# Autodesk Inventor assembly: SpacingStrut
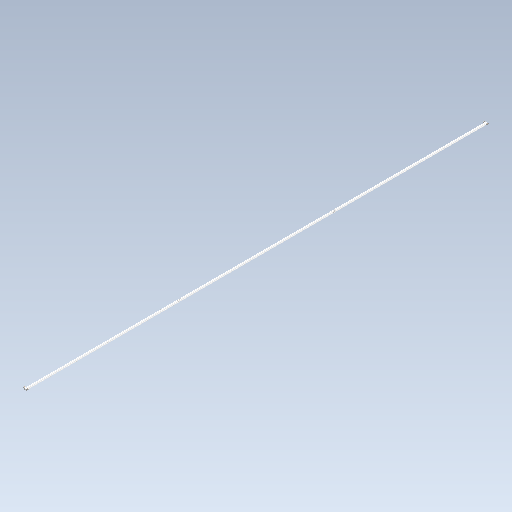
[picture p0: Inventor's stored thumbnail of the model, 512x512]
Saved by Autodesk Inventor 2021 (Build 250183000, 183)
## iProperties
Created: 2021-12-18
Part Number: SpacingStrut
Document SubType Name: Assembly
Designer: Jorian Brusind
Description: Spacing strut used to maintain equal distance between side rails
Author: Jorian Brusind
Revision Number: 1.1
## Documents named in this file (5)
- C:\Users\Jorian Brusind\Documents\GitHub\HyperRail\Inventor Files\SpacingStrut.iam
- C:\Users\Jorian Brusind\Documents\GitHub\PersonalProjects\HyperRail\Inventor Files\8020_Sets\IPT_20_Series\IPT_20_Series\20-2020_1928mm.ipt
- C:\Users\Jorian Brusind\Documents\GitHub\HyperRail\Inventor Files\5537T425_T-SLOTTED FRAMING.ipt
- C:\Users\Jorian Brusind\Documents\GitHub\HyperRail\Inventor Files\8020_Sets\IPT_20_Series\Extra_20_Series\8020_14056m\14056_m.ipt
- C:\Users\Jorian Brusind\Documents\GitHub\PersonalProjects\Inventor Projects\Useful models\Metric bolt\Bolt M5 8mm.ipt
## Components (19 placed, 4 different names)
1. 20-2020_1928mm:1 — Mate:2, Flush:1, Flush:2, Flush:8, Flush:13, Mate:14, Mate:15, Flush:14, Flush:15
2. 20-2020_1928mm:2 — Mate:1, Flush:3, Flush:4, Mate:6, Mate:7, Mate:8, Angle:1, Mate:9, Mate:12, Flush:9, Flush:10, Mate:13, Flush:11, Flush:12
3. 20-2020_1928mm:3 — Mate:1, Mate:2, Flush:1, Flush:2, Flush:3, Flush:4, Mate:4, Mate:5
4. 14056_m:1 — Flush:8, Flush:13, Mate:14, Mate:16, Mate:19
5. 14056_m:2 — Mate:15, Flush:14, Flush:15, Mate:17, Mate:18
6. 14056_m:3 — Mate:12, Flush:9, Flush:10, Mate:20, Mate:22
7. 14056_m:4 — Mate:13, Flush:11, Flush:12, Mate:21, Mate:23
8. Bolt M5 8mm:1 — Mate:16, Mate:19
9. Bolt M5 8mm:2 — Mate:17, Mate:18
10. Bolt M5 8mm:3 — Mate:20, Mate:22
11. Bolt M5 8mm:4 — Mate:21, Mate:23
12. 5537T425_T-SLOTTED FRAMING:1 — Mate:4, Mate:5, Angle:1, Mate:9
13. 5537T425_T-SLOTTED FRAMING:2
14. 5537T425_T-SLOTTED FRAMING:3
15. 5537T425_T-SLOTTED FRAMING:4
16. 5537T425_T-SLOTTED FRAMING:5
17. 5537T425_T-SLOTTED FRAMING:6
18. 5537T425_T-SLOTTED FRAMING:7
19. 5537T425_T-SLOTTED FRAMING:8
## Component patterns: (2 elements), (4 elements, first: 5537T425_T-SLOTTED FRAMING:1), Component Pattern 1:2 (4 elements)
## Relationships (33: Mate 20, Flush 12, Angle 1)
- Mate:1: 20-2020_1928mm:2 ↔ 20-2020_1928mm:3
- Mate:2: 20-2020_1928mm:1 ↔ 20-2020_1928mm:3
- Flush:1: 20-2020_1928mm:1 ↔ 20-2020_1928mm:3
- Flush:2: 20-2020_1928mm:1 ↔ 20-2020_1928mm:3
- Flush:3: 20-2020_1928mm:2 ↔ 20-2020_1928mm:3
- Flush:4: 20-2020_1928mm:2 ↔ 20-2020_1928mm:3
- Mate:4 (2.5 mm): 20-2020_1928mm:3 ↔ 5537T425_T-SLOTTED FRAMING:1
- Mate:5: 20-2020_1928mm:3 ↔ 5537T425_T-SLOTTED FRAMING:1
- Mate:6: 20-2020_1928mm:2
- Mate:7: 20-2020_1928mm:2
- Mate:8: 20-2020_1928mm:2
- Angle:1 (0 deg): 20-2020_1928mm:2 ↔ 5537T425_T-SLOTTED FRAMING:1
- Mate:9 (-1908 mm): 20-2020_1928mm:2 ↔ 5537T425_T-SLOTTED FRAMING:1
- Flush:8: 20-2020_1928mm:1 ↔ 14056_m:1
- Mate:12: 20-2020_1928mm:2 ↔ 14056_m:3
- Flush:9: 20-2020_1928mm:2 ↔ 14056_m:3
- Flush:10: 20-2020_1928mm:2 ↔ 14056_m:3
- Mate:13: 20-2020_1928mm:2 ↔ 14056_m:4
- Flush:11: 20-2020_1928mm:2 ↔ 14056_m:4
- Flush:12: 20-2020_1928mm:2 ↔ 14056_m:4
- Flush:13: 20-2020_1928mm:1 ↔ 14056_m:1
- Mate:14: 20-2020_1928mm:1 ↔ 14056_m:1
- Mate:15: 20-2020_1928mm:1 ↔ 14056_m:2
- Flush:14: 20-2020_1928mm:1 ↔ 14056_m:2
- Flush:15: 20-2020_1928mm:1 ↔ 14056_m:2
- Mate:16: 14056_m:1 ↔ Bolt M5 8mm:1
- Mate:17: 14056_m:2 ↔ Bolt M5 8mm:2
- Mate:18: 14056_m:2 ↔ Bolt M5 8mm:2
- Mate:19: 14056_m:1 ↔ Bolt M5 8mm:1
- Mate:20: 14056_m:3 ↔ Bolt M5 8mm:3
- Mate:21: 14056_m:4 ↔ Bolt M5 8mm:4
- Mate:22: 14056_m:3 ↔ Bolt M5 8mm:3
- Mate:23: 14056_m:4 ↔ Bolt M5 8mm:4
